# Autodesk Inventor assembly: ServoBlock
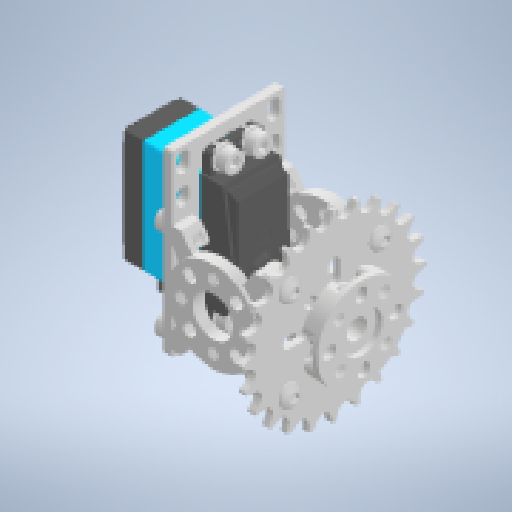
[picture p0: Inventor's stored thumbnail of the model, 512x512]
Saved by Autodesk Inventor 2023 (Build 270158000, 158)
## iProperties
Created: 2022-09-10
Part Number: ServoBlock
Document SubType Name: Assembly
Designer: deli
Author: deli
## Documents named in this file (5)
- C:\Users\deli\OneDrive - Eastside Preparatory School\FTC\8103-power-play\CAD\ServoBlock.iam
- C:\Users\deli\OneDrive - Eastside Preparatory School\FTC\8103-power-play\CAD\FTC-parts\DS3225-SG-Coreless.ipt
- C:\Users\deli\OneDrive - Eastside Preparatory School\FTC\8103-power-play\CAD\FTC-parts\goBILDA\3202-0001-2501.ipt
- C:\Users\deli\OneDrive - Eastside Preparatory School\FTC\8103-power-play\CAD\3311-0014-0024 with 19mm hole.ipt
- C:\Users\deli\OneDrive - Eastside Preparatory School\FTC\8103-power-play\CAD\FTC-parts\goBILDA\2802-0004-0010.ipt
## Components (7 placed, 4 different names)
1. DS3225-SG-Coreless:1 — Mate:1, Mate:2, Angle:1
2. 3202-0001-2501:1 — Mate:1, Mate:2, Angle:1, Mate:6, Mate:7, Mate:8
3. 3311-0014-0024 with 19mm hole:1 — Mate:6, Mate:7, Mate:8, Mate:11, Mate:12, Mate:13, Mate:14, Mate:15, Mate:16
4. 2802-0004-0010:1 — Mate:12
5. 2802-0004-0010:2 — Mate:15, Mate:16
6. 2802-0004-0010:3 — Mate:11, Mate:13
7. 2802-0004-0010:4 — Mate:14
## Relationships (14: Mate 13, Angle 1)
- Mate:1: DS3225-SG-Coreless:1 ↔ 3202-0001-2501:1
- Mate:2: DS3225-SG-Coreless:1 ↔ 3202-0001-2501:1
- Angle:1 (0 deg): DS3225-SG-Coreless:1 ↔ 3202-0001-2501:1
- Mate:6: 3202-0001-2501:1 ↔ 3311-0014-0024 with 19mm hole:1
- Mate:7: 3202-0001-2501:1 ↔ 3311-0014-0024 with 19mm hole:1
- Mate:8: 3202-0001-2501:1 ↔ 3311-0014-0024 with 19mm hole:1
- [Mate]: 3311-0014-0024 with 19mm hole:1 ↔ 2802-0004-0010:4
- [Mate]: 3311-0014-0024 with 19mm hole:1 ↔ 2802-0004-0010:1
- Mate:11: 3311-0014-0024 with 19mm hole:1 ↔ 2802-0004-0010:3
- Mate:12: 3311-0014-0024 with 19mm hole:1 ↔ 2802-0004-0010:1
- Mate:13: 3311-0014-0024 with 19mm hole:1 ↔ 2802-0004-0010:3
- Mate:14: 3311-0014-0024 with 19mm hole:1 ↔ 2802-0004-0010:4
- Mate:15: 3311-0014-0024 with 19mm hole:1 ↔ 2802-0004-0010:2
- Mate:16: 3311-0014-0024 with 19mm hole:1 ↔ 2802-0004-0010:2
